# Autodesk Inventor assembly: am-2878+Banebots+P60+256-11(Fixed)
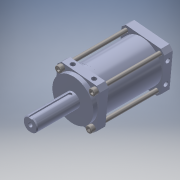
[picture p0: Inventor's stored thumbnail of the model, 180x180]
Saved by Autodesk Inventor 2017 (Build 210142000, 142)
## iProperties
Created: 2015-01-09
Part Number: am-2878+Banebots+P60+256-11(Fixed)
Description: STEP AP214
Document SubType Name: Assembly
Designer: kingb
Sending System: SolidWorks 2014
Preprocessor: SwSTEP 2.0
Title: am-2878 Banebots P60 256-1.STEP
Revision Number: ANY
## Documents named in this file (5)
- C:\Users\kingb\Desktop\CAD\am-2878+Banebots+P60+256-11(Fixed).iam
- C:\Users\kingb\Desktop\CAD\P60 shaft plate and shaft.ipt
- C:\Users\kingb\Desktop\CAD\P60 4-stage ring gear.ipt
- C:\Users\kingb\Desktop\CAD\P60 motor plate.ipt
- C:\Users\kingb\Desktop\CAD\socket head cap screw_ai_HX-SHCS 0.138-32x2.5x1-N.ipt
## Components (7 placed, 7 different names)
1. P60 shaft plate and shaft_1 — Insert:2, Insert:3, Insert:4, Insert:5, Insert:6
2. P60 4-stage ring gear_2 — Insert:1, Insert:2
3. P60 motor plate_3 — Insert:1, Mate:1
4. socket head cap screw_ai_HX-SHCS 0.138-32x2.5x1-N_4 — Insert:6
5. socket head cap screw_ai_HX-SHCS 0.138-32x2.5x1-N_5 — Mate:1, Insert:3
6. socket head cap screw_ai_HX-SHCS 0.138-32x2.5x1-N_6 — Insert:5
7. socket head cap screw_ai_HX-SHCS 0.138-32x2.5x1-N_7 — Insert:4
## Relationships (7: Insert 6, Mate 1)
- Insert:1: P60 4-stage ring gear_2 ↔ P60 motor plate_3
- Insert:2: P60 shaft plate and shaft_1 ↔ P60 4-stage ring gear_2
- Mate:1: P60 motor plate_3 ↔ socket head cap screw_ai_HX-SHCS 0.138-32x2.5x1-N_5
- Insert:3: P60 shaft plate and shaft_1 ↔ socket head cap screw_ai_HX-SHCS 0.138-32x2.5x1-N_5
- Insert:4: P60 shaft plate and shaft_1 ↔ socket head cap screw_ai_HX-SHCS 0.138-32x2.5x1-N_7
- Insert:5: P60 shaft plate and shaft_1 ↔ socket head cap screw_ai_HX-SHCS 0.138-32x2.5x1-N_6
- Insert:6: P60 shaft plate and shaft_1 ↔ socket head cap screw_ai_HX-SHCS 0.138-32x2.5x1-N_4
